# Autodesk Inventor assembly: lightweight carrige v2
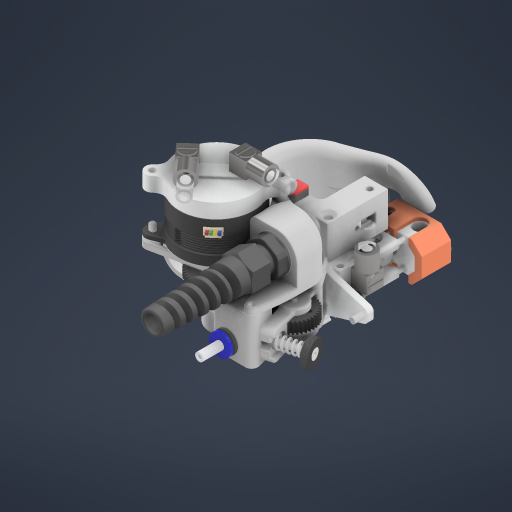
[picture p0: Inventor's stored thumbnail of the model, 512x512]
Saved by Autodesk Inventor 2024.3 (Build 283343000, 343)
## iProperties
Created: 2024-09-28
Part Number: lightweight carrige v2
Document SubType Name: Assembly
Designer: MFil
Author: MFil
## Documents named in this file (33)
- C:\ROBOTYKA\myVORON tridex\Hotend carriges\lightweight carrige v2.iam
- C:\ROBOTYKA\myVORON tridex\Hotend carriges\thin carrige\MGN9H Block.ipt
- C:\ROBOTYKA\myVORON tridex\Hotend carriges\thin carrige\LDO-36STH20-1004AHG.ipt
- C:\ROBOTYKA\myVORON tridex\Hotend carriges\thin carrige\LGX 17T-44T Gear.ipt
- C:\ROBOTYKA\myVORON tridex\Hotend carriges\thin carrige\LGX Hobbed Gear (R).iam
- C:\ROBOTYKA\myVORON tridex\Hotend carriges\thin carrige\MR63ZZ (B).ipt
- C:\ROBOTYKA\myVORON tridex\Hotend carriges\thin carrige\Rocker shaft.ipt
- C:\ROBOTYKA\myVORON tridex\Hotend carriges\thin carrige\Screw M3x8.ipt
- C:\ROBOTYKA\myVORON tridex\Hotend carriges\thin carrige\Rocker screw BASE.iam
- C:\ROBOTYKA\myVORON tridex\Parts\tridex belt a_CPY 4.ipt
- C:\ROBOTYKA\myVORON tridex\Hotend carriges\parts\filament piece.ipt
- C:\ROBOTYKA\myVORON tridex\Parts\IR-endstop-0.4.1.ipt
- C:\ROBOTYKA\myVORON tridex\Hotend carriges\thin carrige\Screw M3x25.ipt
- C:\ROBOTYKA\myVORON tridex\Hotend carriges\parts\6mm hose fitting.ipt
- C:\ROBOTYKA\myVORON tridex\Hotend carriges\parts\ptfe filament guide.ipt
- C:\ROBOTYKA\myVORON tridex\Hotend carriges\parts\colle ptfe guide.ipt
- C:\ROBOTYKA\myVORON tridex\Hotend carriges\parts\mounting plate.ipt
- C:\ROBOTYKA\myVORON tridex\Hotend carriges\parts\belt clip 1.ipt
- C:\ROBOTYKA\myVORON tridex\Hotend carriges\parts\belt clip 1_MIR1.ipt
- C:\ROBOTYKA\myVORON tridex\Hotend carriges\parts\belt clip 2.ipt
- C:\ROBOTYKA\myVORON tridex\Hotend carriges\parts\extruder backplate.ipt
- C:\ROBOTYKA\myVORON tridex\Hotend carriges\parts\extruder front.ipt
- C:\ROBOTYKA\myVORON tridex\Hotend carriges\parts\cpap hose holder.ipt
- C:\ROBOTYKA\myVORON tridex\Hotend carriges\water hotend v2 assembly.iam
- C:\ROBOTYKA\myVORON tridex\Parts\PG7 Flex Gland\PG7 Flex Gland\PG7 Flex Gland.iam
- C:\ROBOTYKA\myVORON tridex\Hotend carriges\20x5 mm spacer.ipt
- C:\ROBOTYKA\myVORON tridex\Hotend carriges\parts\strain relief mount.ipt
- C:\ROBOTYKA\myVORON tridex\Hotend carriges\parts\nema 14 heatsink.ipt
- C:\ROBOTYKA\myVORON tridex\Hotend carriges\parts\nema 14 cooler lid.ipt
- C:\ROBOTYKA\myVORON tridex\Hotend carriges\thin carrige\clicky pcb top.ipt
- C:\ROBOTYKA\myVORON tridex\Hotend carriges\thin carrige\Clicku pcb bottom.ipt
- C:\ROBOTYKA\myVORON tridex\Hotend carriges\thin carrige\Part2.ipt
- C:\ROBOTYKA\myVORON tridex\Hotend carriges\thin carrige\Idler_arm_MIR_MIR3.ipt
## Components (40 placed, 32 different names)
1. MGN9H Block:1 — Mate:36, Tangent:9, Tangent:11, Flush:28, Flush:30, Mate:54, Mate:55
2. Rocker shaft:1 — Flush:49, Mate:108, Mate:110
3. Rocker screw BASE:1 [sub-assembly]
4. tridex belt a_CPY 4:1
5. tridex belt a_CPY 4:2 — Mate:36, Flush:30
6. IR-endstop-0.4.1:1 — Tangent:7, Tangent:8, Tangent:10, Mate:47, Mate:128
7. filament piece:1 — Tangent:7, Tangent:8, Mate:46, Mate:83
8. Screw M3x25:2 — Mate:48, Mate:81, Mate:82, Mate:117
9. LDO-36STH20-1004AHG:1 — Mate:43, Tangent:9, Tangent:11, Mate:48, Mate:49, Mate:50, Flush:51, Tangent:13, Flush:53, Mate:92, Mate:127
10. Screw M3x8:1 — Mate:49, Mate:50, Mate:122
11. MR63ZZ (B):1 — Mate:40, Flush:25, Tangent:10
12. LGX 17T-44T Gear:1 — Mate:41, Flush:24, Flush:25, Mate:43
13. MR63ZZ (B):2 — Mate:40, Mate:41, Flush:24, Mate:91
14. 6mm hose fitting:1 — Flush:19, Mate:96
15. 6mm hose fitting:2 — Flush:19
16. ptfe filament guide:1 — Mate:85
17. colle ptfe guide:1 — Mate:46, Mate:47
18. mounting plate:1 — Flush:28, Mate:51, Mate:54, Mate:55, Mate:62, Flush:50, Mate:84, Mate:87
19. belt clip 1:1 — Mate:51, Flush:32, Mate:65, Mate:102, Mate:103, Flush:106, Flush:108
20. Screw M3x25:4 — Flush:31
21. Screw M3x25:5 — Flush:31, Mate:62, Mate:102
22. belt clip 1_MIR1:1
23. belt clip 2:1 — Flush:32, Mate:65, Mate:103
24. extruder backplate:1 — Mate:89, Mate:91, Mate:92, Mate:117
25. extruder front:1 — Mate:81, Flush:49, Flush:50, Mate:82, Mate:83, Tangent:14, Mate:89, Mate:110, Mate:112, Mate:113, Mate:114, Mate:116, Mate:128
26. 6mm hose fitting:3 — Flush:36, Mate:124
27. 6mm hose fitting:4 — Flush:36, Mate:125, Mate:126
28. cpap hose holder:1
29. water hotend v2 assembly:1 [sub-assembly] — Mate:84, Mate:85, Mate:96, Mate:106
30. PG7 Flex Gland:1 [sub-assembly] — Mate:87, Tangent:13, Tangent:14
31. 20x5 mm spacer:1 — Flush:51, Mate:123, Mate:127
32. strain relief mount:1
33. nema 14 heatsink:1 — Flush:53, Mate:88, Mate:119, Mate:120
34. nema 14 cooler lid:1 — Mate:88, Mate:119, Mate:120, Mate:122, Mate:123, Mate:124, Mate:125, Mate:126
35. clicky pcb top:1 — Flush:54, Mate:99, Mate:101, Flush:106, Mate:106
36. Clicku pcb bottom:1 — Flush:54, Mate:99, Mate:101
37. Part2:1 — Flush:108
38. Idler_arm_MIR_MIR3:1 — Mate:108, Mate:111, Mate:114, Mate:115, Mate:116
39. LGX Hobbed Gear (R):1 [sub-assembly] — Mate:112, Mate:113
40. LGX Hobbed Gear (R):2 [sub-assembly] — Mate:111, Mate:115
## Relationships (73: Mate 49, Flush 17, Tangent 7)
- [Flush]: tridex belt a_CPY 4:1 ↔ tridex belt a_CPY 4:2
- [Mate] (2.5 mm): tridex belt a_CPY 4:1 ↔ tridex belt a_CPY 4:2
- [Flush]: tridex belt a_CPY 4:1 ↔ tridex belt a_CPY 4:2
- Flush:19: 6mm hose fitting:1 ↔ 6mm hose fitting:2
- Tangent:7 (0.525 mm): IR-endstop-0.4.1:1 ↔ filament piece:1
- Tangent:8 (0.075 mm): IR-endstop-0.4.1:1 ↔ filament piece:1
- Mate:36 (3.3 mm): MGN9H Block:1 ↔ tridex belt a_CPY 4:2
- Mate:40: MR63ZZ (B):1 ↔ MR63ZZ (B):2
- Mate:41: LGX 17T-44T Gear:1 ↔ MR63ZZ (B):2
- Flush:24: LGX 17T-44T Gear:1 ↔ MR63ZZ (B):2
- Flush:25: MR63ZZ (B):1 ↔ LGX 17T-44T Gear:1
- Mate:43 (13.5 mm): LDO-36STH20-1004AHG:1 ↔ LGX 17T-44T Gear:1
- Tangent:9 (6 mm): MGN9H Block:1 ↔ LDO-36STH20-1004AHG:1
- Tangent:10 (2 mm): IR-endstop-0.4.1:1 ↔ MR63ZZ (B):1
- Tangent:11 (6 mm): MGN9H Block:1 ↔ LDO-36STH20-1004AHG:1
- Mate:46: filament piece:1 ↔ colle ptfe guide:1
- Mate:47 (1 mm): IR-endstop-0.4.1:1 ↔ colle ptfe guide:1
- Flush:28: MGN9H Block:1 ↔ mounting plate:1
- Mate:48: Screw M3x25:2 ↔ LDO-36STH20-1004AHG:1
- Mate:49: LDO-36STH20-1004AHG:1 ↔ Screw M3x8:1
- Mate:50 (3 mm): LDO-36STH20-1004AHG:1 ↔ Screw M3x8:1
- Flush:30 (7.994 mm): MGN9H Block:1 ↔ tridex belt a_CPY 4:2
- Mate:51: mounting plate:1 ↔ belt clip 1:1
- Mate:54: MGN9H Block:1 ↔ mounting plate:1
- Mate:55: MGN9H Block:1 ↔ mounting plate:1
- Flush:31: Screw M3x25:4 ↔ Screw M3x25:5
- Mate:62: mounting plate:1 ↔ Screw M3x25:5
- Flush:32: belt clip 1:1 ↔ belt clip 2:1
- Mate:65 (0.2 mm): belt clip 1:1 ↔ belt clip 2:1
- Flush:36: 6mm hose fitting:3 ↔ 6mm hose fitting:4
- Mate:81: Screw M3x25:2 ↔ extruder front:1
- Flush:49: Rocker shaft:1 ↔ extruder front:1
- Flush:50 (-3 mm): mounting plate:1 ↔ extruder front:1
- Mate:82: Screw M3x25:2 ↔ extruder front:1
- Mate:83: filament piece:1 ↔ extruder front:1
- Mate:84: mounting plate:1 ↔ water hotend v2 assembly:1
- Mate:85: ptfe filament guide:1 ↔ water hotend v2 assembly:1
- Flush:51: LDO-36STH20-1004AHG:1 ↔ 20x5 mm spacer:1
- Mate:87 (15 mm): mounting plate:1 ↔ PG7 Flex Gland:1
- Tangent:13 (3 mm): LDO-36STH20-1004AHG:1 ↔ PG7 Flex Gland:1
- Tangent:14 (6 mm): extruder front:1 ↔ PG7 Flex Gland:1
- Flush:53: LDO-36STH20-1004AHG:1 ↔ nema 14 heatsink:1
- Mate:88: nema 14 heatsink:1 ↔ nema 14 cooler lid:1
- Mate:89: extruder backplate:1 ↔ extruder front:1
- Mate:91: MR63ZZ (B):2 ↔ extruder backplate:1
- Mate:92: LDO-36STH20-1004AHG:1 ↔ extruder backplate:1
- Mate:96: 6mm hose fitting:1 ↔ water hotend v2 assembly:1
- Flush:54: clicky pcb top:1 ↔ Clicku pcb bottom:1
- Mate:99: clicky pcb top:1 ↔ Clicku pcb bottom:1
- Mate:101: clicky pcb top:1 ↔ Clicku pcb bottom:1
- Mate:102: belt clip 1:1 ↔ Screw M3x25:5
- Mate:103: belt clip 1:1 ↔ belt clip 2:1
- Flush:106 (1.361 mm): belt clip 1:1 ↔ clicky pcb top:1
- Mate:106 (13.95 mm): water hotend v2 assembly:1 ↔ clicky pcb top:1
- Mate:108: Rocker shaft:1 ↔ Idler_arm_MIR_MIR3:1
- Mate:110: Rocker shaft:1 ↔ extruder front:1
- Mate:111: Idler_arm_MIR_MIR3:1 ↔ LGX Hobbed Gear (R):2
- Mate:112: extruder front:1 ↔ LGX Hobbed Gear (R):1
- Mate:113: extruder front:1 ↔ LGX Hobbed Gear (R):1
- Mate:114 (0.2 mm): extruder front:1 ↔ Idler_arm_MIR_MIR3:1
- Mate:115 (0.5 mm): Idler_arm_MIR_MIR3:1 ↔ LGX Hobbed Gear (R):2
- Mate:116: extruder front:1 ↔ Idler_arm_MIR_MIR3:1
- Mate:117: Screw M3x25:2 ↔ extruder backplate:1
- Flush:108: belt clip 1:1 ↔ Part2:1
- Mate:119: nema 14 heatsink:1 ↔ nema 14 cooler lid:1
- Mate:120: nema 14 heatsink:1 ↔ nema 14 cooler lid:1
- Mate:122: Screw M3x8:1 ↔ nema 14 cooler lid:1
- Mate:123: 20x5 mm spacer:1 ↔ nema 14 cooler lid:1
- Mate:124: 6mm hose fitting:3 ↔ nema 14 cooler lid:1
- Mate:125: 6mm hose fitting:4 ↔ nema 14 cooler lid:1
- Mate:126: 6mm hose fitting:4 ↔ nema 14 cooler lid:1
- Mate:127: LDO-36STH20-1004AHG:1 ↔ 20x5 mm spacer:1
- Mate:128 (0.2 mm): IR-endstop-0.4.1:1 ↔ extruder front:1
